# Autodesk Inventor assembly: 0001001
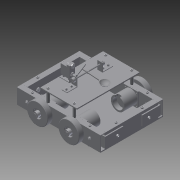
[picture p0: Inventor's stored thumbnail of the model, 180x180]
Saved by Autodesk Inventor 2015 (Build 190159000, 159)
## iProperties
Created: 2015-05-31
Part Number: 0001001
Document SubType Name: Assembly
Designer: Wesley
Author: Wesley
## Documents named in this file (24)
- C:\Users\Wesley\Documents\GitHub\EngineeringFinal\Engineering\Engineering Documentation\0001__\0001001.iam
- C:\Users\Wesley\Documents\GitHub\EngineeringFinal\Engineering\Engineering Documentation\0001__\000101-1.ipt
- C:\Users\Wesley\Documents\GitHub\EngineeringFinal\Engineering\Engineering Documentation\0001__\000101-2.ipt
- C:\Users\Wesley\Documents\GitHub\EngineeringFinal\Engineering\Engineering Documentation\0001__\000103.ipt
- C:\Users\Wesley\Documents\GitHub\EngineeringFinal\Engineering\Engineering Documentation\0001__\000102.ipt
- C:\Users\Wesley\Documents\GitHub\EngineeringFinal\Engineering\Engineering Documentation\0001__\000104.ipt
- C:\Users\Wesley\Documents\GitHub\EngineeringFinal\Engineering\Engineering Documentation\0001__\000107.ipt
- C:\Users\Wesley\Documents\GitHub\EngineeringFinal\Engineering\Engineering Documentation\0001__\000108.ipt
- C:\Users\Wesley\Documents\GitHub\EngineeringFinal\Engineering\Engineering Documentation\0001__\000109.ipt
- C:\Users\Wesley\Documents\GitHub\EngineeringFinal\Engineering\Engineering Documentation\0001__\000110.ipt
- C:\Users\Wesley\Documents\GitHub\EngineeringFinal\Engineering\Engineering Documentation\0001__\000105-1.ipt
- C:\Users\Wesley\Documents\GitHub\EngineeringFinal\Engineering\Engineering Documentation\0001__\000106.ipt
- C:\Users\Wesley\Documents\GitHub\EngineeringFinal\Engineering\Engineering Documentation\0001__\000105-2.ipt
- C:\Users\Wesley\Documents\GitHub\EngineeringFinal\Engineering\Engineering Documentation\0002__\000202.ipt
- C:\Users\Wesley\Documents\GitHub\EngineeringFinal\Engineering\Engineering Documentation\0002__\000201.ipt
- C:\Users\Wesley\Documents\GitHub\EngineeringFinal\Engineering\Engineering Documentation\0002__\000204.ipt
- C:\Users\Wesley\Documents\GitHub\EngineeringFinal\Engineering\Engineering Documentation\0002__\000203.ipt
- C:\Users\Wesley\Documents\GitHub\EngineeringFinal\Engineering\Engineering Documentation\0002__\000205.ipt
- C:\Users\Wesley\Documents\GitHub\EngineeringFinal\Engineering\Engineering Documentation\0002__\000208.ipt
- C:\Users\Wesley\Documents\GitHub\EngineeringFinal\Engineering\Engineering Documentation\0002__\000206.ipt
- C:\Users\Wesley\Documents\GitHub\EngineeringFinal\Engineering\Engineering Documentation\0002__\000207.ipt
- C:\Users\Wesley\Documents\GitHub\EngineeringFinal\Engineering\Engineering Documentation\0002__\000210-1.ipt
- C:\Users\Wesley\Documents\GitHub\EngineeringFinal\Engineering\Engineering Documentation\0002__\000210-2.ipt
- C:\Users\Wesley\Documents\GitHub\EngineeringFinal\Engineering\Engineering Documentation\0002__\000209.ipt
## Components (97 placed, 23 different names)
1. 000101-1:1 — Mate:4, Mate:5, Mate:6, Flush:3, Mate:8, Mate:14, Mate:20, Mate:33, Mate:34, Flush:7, Mate:35, Mate:36, Flush:8, Mate:58, Mate:59, Mate:69, Mate:70, Mate:72, Mate:73, Mate:74, Mate:76, Mate:105, Mate:106, Mate:107, Mate:108, Mate:137, Mate:140
2. 000101-1:2 — Mate:1, Mate:2, Mate:3, Mate:7, Flush:1, Flush:2, Flush:4, Mate:11, Mate:18, Mate:29, Mate:30, Flush:5, Mate:31, Mate:32, Flush:6, Mate:46, Mate:52, Mate:85, Mate:86, Mate:88, Mate:89, Mate:90, Mate:92, Mate:113, Mate:114, Mate:115, Mate:116, Mate:131, Mate:133, Mate:134
3. 000101-2:1 — Flush:3, Flush:4, Mate:8, Mate:15, Mate:16, Mate:17, Mate:19, Mate:80, Mate:81, Mate:84, Mate:109, Mate:110, Mate:111, Mate:112
4. 000101-2:2 — Mate:7, Flush:1, Flush:2, Mate:9, Mate:10, Mate:12, Mate:13, Mate:64, Mate:68, Mate:101, Mate:102, Mate:103, Mate:104
5. 000103:1 — Mate:1, Mate:2, Mate:3, Mate:4, Mate:5, Mate:6, Mate:117, Mate:118, Mate:119, Mate:120, Mate:121, Mate:122, Mate:123, Mate:124, Mate:129, Mate:130, Mate:132, Mate:135, Mate:136, Mate:138, Mate:139
6. 000102:1 — Mate:12, Mate:13, Mate:14, Mate:65, Mate:66
7. 000102:2 — Mate:16, Mate:19, Mate:20, Mate:77, Mate:78
8. 000102:3 — Mate:15, Mate:17, Mate:18, Mate:82
9. 000102:4 — Mate:9, Mate:10, Mate:11, Mate:61, Mate:62
10. 000104:1 — Mate:45, Mate:46, Mate:47, Mate:48
11. 000104:2 — Mate:49, Mate:50, Mate:51, Mate:52
12. 000104:3 — Mate:53, Mate:54, Mate:57, Mate:58
13. 000104:4 — Mate:55, Mate:56, Mate:59, Mate:60
14. 000107:1 — Mate:47, Mate:48
15. 000107:2 — Mate:55, Mate:56
16. 000107:3 — Mate:53, Mate:54
17. 000107:4 — Mate:49, Mate:50
18. 000108:1 — Mate:43, Mate:44
19. 000108:2 — Mate:39, Mate:40
20. 000108:3 — Mate:41, Mate:42
21. 000108:4 — Mate:37, Mate:38
22. 000109:1 — Mate:21, Mate:22, Mate:39
23. 000110:1 — Mate:21, Mate:22, Mate:31, Mate:32, Flush:6, Mate:40, Mate:45
24. 000109:2 — Mate:23, Mate:24, Mate:41
25. 000110:2 — Mate:23, Mate:24, Mate:33, Mate:34, Flush:7, Mate:42, Mate:60
26. 000109:3 — Mate:25, Mate:26, Mate:43
27. 000110:3 — Mate:25, Mate:26, Mate:35, Mate:36, Flush:8, Mate:44, Mate:57
28. 000109:4 — Mate:27, Mate:28, Mate:38
29. 000110:4 — Mate:27, Mate:28, Mate:29, Mate:30, Flush:5, Mate:37, Mate:51
30. 000105-1:1 — Mate:65, Mate:66, Mate:67
31. 000105-1:2 — Mate:61, Mate:62, Mate:63
32. 000105-1:3 — Mate:69, Mate:70, Mate:71
33. 000105-1:4 — Mate:73, Mate:74, Mate:75
34. 000105-1:5 — Mate:77, Mate:78, Mate:79
35. 000105-1:6 — Mate:81, Mate:82, Mate:83
36. 000105-1:7 — Mate:85, Mate:86, Mate:87
37. 000105-1:8 — Mate:89, Mate:90, Mate:91
38. 000106:1 — Mate:75, Mate:76
39. 000106:2 — Mate:63, Mate:64
40. 000106:3 — Mate:67, Mate:68
41. 000106:4 — Mate:71, Mate:72
42. 000106:5 — Mate:79, Mate:80
43. 000106:6 — Mate:83, Mate:84
44. 000106:7 — Mate:87, Mate:88
45. 000106:8 — Mate:91, Mate:92
46. 000105-2:1 — Mate:100, Mate:101, Mate:102
47. 000105-2:2 — Mate:99, Mate:103, Mate:104
48. 000105-2:3 — Mate:98, Mate:105, Mate:106
49. 000105-2:4 — Mate:97, Mate:109, Mate:110
50. 000105-2:5 — Mate:96, Mate:115, Mate:116
51. 000105-2:6 — Mate:95, Mate:113, Mate:114
52. 000105-2:7 — Mate:94, Mate:111, Mate:112
53. 000105-2:8 — Mate:93, Mate:107, Mate:108
54. 000106:9 — Mate:95, Mate:120
55. 000106:10 — Mate:96, Mate:119
56. 000106:11 — Mate:97, Mate:124
57. 000106:12 — Mate:98, Mate:118
58. 000106:13 — Mate:99, Mate:121
59. 000106:14 — Mate:100, Mate:117
60. 000106:15 — Mate:93, Mate:123
61. 000106:16 — Mate:94, Mate:122
62. 000202:1 — Mate:128, Mate:140
63. 000202:2 — Mate:127, Mate:137, Mate:141
64. 000202:3 — Mate:126, Mate:134, Mate:142
65. 000202:4 — Mate:125, Mate:131, Mate:143
66. 000105-2:9 — Mate:126, Mate:132, Mate:133
67. 000105-2:10 — Mate:128, Mate:138, Mate:139
68. 000105-2:11 — Mate:127, Mate:135, Mate:136
69. 000105-2:12 — Mate:125, Mate:129, Mate:130
70. 000201:1 — Mate:141, Mate:142, Mate:143, Mate:144, Mate:145, Mate:146, Mate:147, Mate:148, Mate:149, Mate:153, Mate:154, Mate:155, Mate:161, Mate:162, Mate:163, Mate:164, Mate:165, Mate:166, Mate:167, Mate:168, Mate:178, Mate:181, Mate:184, Mate:187, Mate:195, Mate:199
71. 000204:1 — Mate:144, Mate:145, Mate:146, Flush:9, Mate:176, Mate:177, Mate:179, Mate:180, Mate:203
72. 000204:2 — Mate:147, Mate:148, Mate:149, Mate:150, Mate:152, Mate:194, Mate:196, Mate:197, Mate:198, Mate:201
73. 000203:1 — Mate:150, Flush:9, Mate:151, Mate:200, Mate:202
74. 000205:1 — Mate:151, Mate:152
75. 000208:1 — Mate:153, Mate:154, Mate:155, Mate:182, Mate:183, Mate:185, Mate:186, Mate:188, Mate:189, Mate:190, Mate:191, Mate:193
76. 000206:2 — Mate:160, Flush:10, Mate:189, Mate:190, Mate:191, Mate:192
77. 000207:1 — Mate:160, Flush:10
78. 000210-1:1 — Mate:165, Mate:167
79. 000210-1:2 — Mate:163, Mate:164
80. 000210-1:3 — Mate:166, Mate:168
81. 000210-1:4 — Mate:161, Mate:162
82. 000210-2:1 — Mate:175, Mate:194, Mate:196
83. 000210-2:2 — Mate:174, Mate:197, Mate:198
84. 000210-2:3 — Mate:173, Mate:176, Mate:177
85. 000210-2:4 — Mate:172, Mate:182, Mate:183
86. 000210-2:5 — Mate:171, Mate:188, Mate:192
87. 000210-2:6 — Mate:170, Mate:185, Mate:186
88. 000210-2:7 — Mate:169, Mate:179, Mate:180
89. 000106:17 — Mate:169, Mate:181
90. 000106:18 — Mate:170, Mate:187
91. 000106:19 — Mate:173, Mate:178
92. 000106:20 — Mate:171, Mate:193
93. 000106:21 — Mate:172, Mate:184
94. 000106:22 — Mate:175, Mate:195
95. 000106:23 — Mate:174, Mate:199
96. 000209:1 — Mate:200, Mate:201
97. 000209:2 — Mate:202, Mate:203
## Relationships (209: Mate 199, Flush 10)
- Mate:1: 000101-1:2 ↔ 000103:1
- Mate:2: 000101-1:2 ↔ 000103:1
- Mate:3: 000101-1:2 ↔ 000103:1
- Mate:4: 000101-1:1 ↔ 000103:1
- Mate:5: 000101-1:1 ↔ 000103:1
- Mate:6: 000101-1:1 ↔ 000103:1
- Mate:7: 000101-1:2 ↔ 000101-2:2
- Flush:1: 000101-1:2 ↔ 000101-2:2
- Flush:2: 000101-1:2 ↔ 000101-2:2
- Flush:3: 000101-1:1 ↔ 000101-2:1
- Flush:4: 000101-1:2 ↔ 000101-2:1
- Mate:8: 000101-1:1 ↔ 000101-2:1
- Mate:9: 000101-2:2 ↔ 000102:4
- Mate:10: 000101-2:2 ↔ 000102:4
- Mate:11: 000101-1:2 ↔ 000102:4
- Mate:12: 000101-2:2 ↔ 000102:1
- Mate:13: 000101-2:2 ↔ 000102:1
- Mate:14: 000101-1:1 ↔ 000102:1
- Mate:15: 000101-2:1 ↔ 000102:3
- Mate:16: 000101-2:1 ↔ 000102:2
- Mate:17: 000101-2:1 ↔ 000102:3
- Mate:18: 000101-1:2 ↔ 000102:3
- Mate:19: 000101-2:1 ↔ 000102:2
- Mate:20: 000101-1:1 ↔ 000102:2
- Mate:21: 000109:1 ↔ 000110:1
- Mate:22: 000109:1 ↔ 000110:1
- Mate:23: 000109:2 ↔ 000110:2
- Mate:24: 000109:2 ↔ 000110:2
- Mate:25: 000109:3 ↔ 000110:3
- Mate:26: 000109:3 ↔ 000110:3
- Mate:27: 000109:4 ↔ 000110:4
- Mate:28: 000109:4 ↔ 000110:4
- Mate:29: 000101-1:2 ↔ 000110:4
- Mate:30: 000101-1:2 ↔ 000110:4
- Flush:5: 000101-1:2 ↔ 000110:4
- Mate:31: 000101-1:2 ↔ 000110:1
- Mate:32: 000101-1:2 ↔ 000110:1
- Flush:6: 000101-1:2 ↔ 000110:1
- Mate:33: 000101-1:1 ↔ 000110:2
- Mate:34: 000101-1:1 ↔ 000110:2
- Flush:7: 000101-1:1 ↔ 000110:2
- Mate:35: 000101-1:1 ↔ 000110:3
- Mate:36: 000101-1:1 ↔ 000110:3
- Flush:8: 000101-1:1 ↔ 000110:3
- Mate:37: 000108:4 ↔ 000110:4
- Mate:38: 000108:4 ↔ 000109:4
- Mate:39: 000108:2 ↔ 000109:1
- Mate:40: 000108:2 ↔ 000110:1
- Mate:41: 000108:3 ↔ 000109:2
- Mate:42: 000108:3 ↔ 000110:2
- Mate:43: 000108:1 ↔ 000109:3
- Mate:44: 000108:1 ↔ 000110:3
- Mate:45: 000104:1 ↔ 000110:1
- Mate:46 (1.27 mm): 000101-1:2 ↔ 000104:1
- Mate:47: 000104:1 ↔ 000107:1
- Mate:48: 000104:1 ↔ 000107:1
- Mate:49: 000104:2 ↔ 000107:4
- Mate:50: 000104:2 ↔ 000107:4
- Mate:51: 000104:2 ↔ 000110:4
- Mate:52 (1.27 mm): 000101-1:2 ↔ 000104:2
- Mate:53: 000104:3 ↔ 000107:3
- Mate:54: 000104:3 ↔ 000107:3
- Mate:55: 000104:4 ↔ 000107:2
- Mate:56: 000104:4 ↔ 000107:2
- Mate:57: 000104:3 ↔ 000110:3
- Mate:58 (1.27 mm): 000101-1:1 ↔ 000104:3
- Mate:59 (1.27 mm): 000101-1:1 ↔ 000104:4
- Mate:60: 000104:4 ↔ 000110:2
- Mate:61: 000102:4 ↔ 000105-1:2
- Mate:62: 000102:4 ↔ 000105-1:2
- Mate:63: 000105-1:2 ↔ 000106:2
- Mate:64: 000101-2:2 ↔ 000106:2
- Mate:65: 000102:1 ↔ 000105-1:1
- Mate:66: 000102:1 ↔ 000105-1:1
- Mate:67: 000105-1:1 ↔ 000106:3
- Mate:68: 000101-2:2 ↔ 000106:3
- Mate:69: 000101-1:1 ↔ 000105-1:3
- Mate:70: 000101-1:1 ↔ 000105-1:3
- Mate:71: 000105-1:3 ↔ 000106:4
- Mate:72: 000101-1:1 ↔ 000106:4
- Mate:73: 000101-1:1 ↔ 000105-1:4
- Mate:74: 000101-1:1 ↔ 000105-1:4
- Mate:75: 000105-1:4 ↔ 000106:1
- Mate:76: 000101-1:1 ↔ 000106:1
- Mate:77: 000102:2 ↔ 000105-1:5
- Mate:78: 000102:2 ↔ 000105-1:5
- Mate:79: 000105-1:5 ↔ 000106:5
- Mate:80: 000101-2:1 ↔ 000106:5
- Mate:81: 000101-2:1 ↔ 000105-1:6
- Mate:82: 000102:3 ↔ 000105-1:6
- Mate:83: 000105-1:6 ↔ 000106:6
- Mate:84: 000101-2:1 ↔ 000106:6
- Mate:85: 000101-1:2 ↔ 000105-1:7
- Mate:86: 000101-1:2 ↔ 000105-1:7
- Mate:87: 000105-1:7 ↔ 000106:7
- Mate:88: 000101-1:2 ↔ 000106:7
- Mate:89: 000101-1:2 ↔ 000105-1:8
- Mate:90: 000101-1:2 ↔ 000105-1:8
- Mate:91: 000105-1:8 ↔ 000106:8
- Mate:92: 000101-1:2 ↔ 000106:8
- Mate:93: 000105-2:8 ↔ 000106:15
- Mate:94: 000105-2:7 ↔ 000106:16
- Mate:95: 000105-2:6 ↔ 000106:9
- Mate:96: 000105-2:5 ↔ 000106:10
- Mate:97: 000105-2:4 ↔ 000106:11
- Mate:98: 000105-2:3 ↔ 000106:12
- Mate:99: 000105-2:2 ↔ 000106:13
- Mate:100: 000105-2:1 ↔ 000106:14
- Mate:101: 000101-2:2 ↔ 000105-2:1
- Mate:102: 000101-2:2 ↔ 000105-2:1
- Mate:103: 000101-2:2 ↔ 000105-2:2
- Mate:104: 000101-2:2 ↔ 000105-2:2
- Mate:105: 000101-1:1 ↔ 000105-2:3
- Mate:106: 000101-1:1 ↔ 000105-2:3
- Mate:107: 000101-1:1 ↔ 000105-2:8
- Mate:108: 000101-1:1 ↔ 000105-2:8
- Mate:109: 000101-2:1 ↔ 000105-2:4
- Mate:110: 000101-2:1 ↔ 000105-2:4
- Mate:111: 000101-2:1 ↔ 000105-2:7
- Mate:112: 000101-2:1 ↔ 000105-2:7
- Mate:113: 000101-1:2 ↔ 000105-2:6
- Mate:114: 000101-1:2 ↔ 000105-2:6
- Mate:115: 000101-1:2 ↔ 000105-2:5
- Mate:116: 000101-1:2 ↔ 000105-2:5
- Mate:117: 000103:1 ↔ 000106:14
- Mate:118: 000103:1 ↔ 000106:12
- Mate:119: 000103:1 ↔ 000106:10
- Mate:120: 000103:1 ↔ 000106:9
- Mate:121: 000103:1 ↔ 000106:13
- Mate:122: 000103:1 ↔ 000106:16
- Mate:123: 000103:1 ↔ 000106:15
- Mate:124: 000103:1 ↔ 000106:11
- Mate:125: 000202:4 ↔ 000105-2:12
- Mate:126: 000202:3 ↔ 000105-2:9
- Mate:127: 000202:2 ↔ 000105-2:11
- Mate:128: 000202:1 ↔ 000105-2:10
- Mate:129: 000103:1 ↔ 000105-2:12
- Mate:130: 000103:1 ↔ 000105-2:12
- Mate:131: 000101-1:2 ↔ 000202:4
- Mate:132: 000103:1 ↔ 000105-2:9
- Mate:133: 000101-1:2 ↔ 000105-2:9
- Mate:134: 000101-1:2 ↔ 000202:3
- Mate:135: 000103:1 ↔ 000105-2:11
- Mate:136: 000103:1 ↔ 000105-2:11
- Mate:137: 000101-1:1 ↔ 000202:2
- Mate:138: 000103:1 ↔ 000105-2:10
- Mate:139: 000103:1 ↔ 000105-2:10
- Mate:140: 000101-1:1 ↔ 000202:1
- Mate:141: 000202:2 ↔ 000201:1
- Mate:142: 000202:3 ↔ 000201:1
- Mate:143: 000202:4 ↔ 000201:1
- Mate:144: 000201:1 ↔ 000204:1
- Mate:145: 000201:1 ↔ 000204:1
- Mate:146: 000201:1 ↔ 000204:1
- Mate:147: 000201:1 ↔ 000204:2
- Mate:148: 000201:1 ↔ 000204:2
- Mate:149: 000201:1 ↔ 000204:2
- Mate:150: 000204:2 ↔ 000203:1
- Flush:9 (-6.35 mm): 000204:1 ↔ 000203:1
- Mate:151: 000203:1 ↔ 000205:1
- Mate:152 (28.575 mm): 000204:2 ↔ 000205:1
- Mate:153: 000201:1 ↔ 000208:1
- Mate:154: 000201:1 ↔ 000208:1
- Mate:155: 000201:1 ↔ 000208:1
- Mate:160: 000206:2 ↔ 000207:1
- Flush:10: 000206:2 ↔ 000207:1
- Mate:161: 000201:1 ↔ 000210-1:4
- Mate:162: 000201:1 ↔ 000210-1:4
- Mate:163: 000201:1 ↔ 000210-1:2
- Mate:164: 000201:1 ↔ 000210-1:2
- Mate:165: 000201:1 ↔ 000210-1:1
- Mate:166: 000201:1 ↔ 000210-1:3
- Mate:167: 000201:1 ↔ 000210-1:1
- Mate:168: 000201:1 ↔ 000210-1:3
- Mate:169: 000210-2:7 ↔ 000106:17
- Mate:170: 000210-2:6 ↔ 000106:18
- Mate:171: 000210-2:5 ↔ 000106:20
- Mate:172: 000210-2:4 ↔ 000106:21
- Mate:173: 000210-2:3 ↔ 000106:19
- Mate:174: 000210-2:2 ↔ 000106:23
- Mate:175: 000210-2:1 ↔ 000106:22
- Mate:176: 000204:1 ↔ 000210-2:3
- Mate:177: 000204:1 ↔ 000210-2:3
- Mate:178: 000201:1 ↔ 000106:19
- Mate:179: 000204:1 ↔ 000210-2:7
- Mate:180: 000204:1 ↔ 000210-2:7
- Mate:181: 000201:1 ↔ 000106:17
- Mate:182: 000208:1 ↔ 000210-2:4
- Mate:183: 000208:1 ↔ 000210-2:4
- Mate:184: 000201:1 ↔ 000106:21
- Mate:185: 000208:1 ↔ 000210-2:6
- Mate:186: 000208:1 ↔ 000210-2:6
- Mate:187: 000201:1 ↔ 000106:18
- Mate:188: 000208:1 ↔ 000210-2:5
- Mate:189: 000208:1 ↔ 000206:2
- Mate:190: 000208:1 ↔ 000206:2
- Mate:191: 000208:1 ↔ 000206:2
- Mate:192: 000206:2 ↔ 000210-2:5
- Mate:193: 000208:1 ↔ 000106:20
- Mate:194: 000204:2 ↔ 000210-2:1
- Mate:195: 000201:1 ↔ 000106:22
- Mate:196: 000204:2 ↔ 000210-2:1
- Mate:197: 000204:2 ↔ 000210-2:2
- Mate:198: 000204:2 ↔ 000210-2:2
- Mate:199: 000201:1 ↔ 000106:23
- Mate:200: 000203:1 ↔ 000209:1
- Mate:201: 000204:2 ↔ 000209:1
- Mate:202: 000203:1 ↔ 000209:2
- Mate:203: 000204:1 ↔ 000209:2
